# Autodesk Inventor assembly: paddlewheel_assem
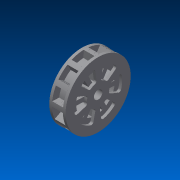
[picture p0: Inventor's stored thumbnail of the model, 180x180]
Saved by Autodesk Inventor 2019 (Build 230136000, 136)
## iProperties
Created: 2018-08-23
Part Number: paddlewheel_assem
Document SubType Name: Assembly
Designer: Kitte_X
Author: Kitte_X
## Documents named in this file (3)
- C:\Users\Kitte_X\Documents\Inventor\paddlewheel_assem.iam
- C:\Users\Kitte_X\Documents\Inventor\paddlewheel_inner.ipt
- C:\Users\Kitte_X\Documents\Inventor\paddlewheel_outer.ipt
## Components (6 placed, 2 different names)
1. paddlewheel_inner:1 — Mate:14, Mate:18, Flush:14, Mate:21, Mate:22
2. paddlewheel_outer:1 — Flush:12, Mate:21, Mate:22, Mate:23, Mate:25, Flush:17
3. paddlewheel_inner:2 — Flush:13, Mate:14, Mate:15, Mate:18, Mate:19, Flush:14, Flush:15
4. paddlewheel_outer:2 — Flush:12, Flush:13, Mate:23, Mate:24
5. paddlewheel_inner:3 — Mate:16, Mate:20, Flush:16, Mate:24
6. paddlewheel_inner:4 — Mate:15, Mate:16, Mate:19, Mate:20, Flush:15, Flush:16
## Relationships (17: Mate 11, Flush 6)
- Flush:12: paddlewheel_outer:1 ↔ paddlewheel_outer:2
- Flush:13: paddlewheel_inner:2 ↔ paddlewheel_outer:2
- Mate:14: paddlewheel_inner:1 ↔ paddlewheel_inner:2
- Mate:15: paddlewheel_inner:2 ↔ paddlewheel_inner:4
- Mate:16: paddlewheel_inner:3 ↔ paddlewheel_inner:4
- Mate:18: paddlewheel_inner:1 ↔ paddlewheel_inner:2
- Mate:19: paddlewheel_inner:2 ↔ paddlewheel_inner:4
- Mate:20: paddlewheel_inner:3 ↔ paddlewheel_inner:4
- Flush:14: paddlewheel_inner:1 ↔ paddlewheel_inner:2
- Flush:15: paddlewheel_inner:2 ↔ paddlewheel_inner:4
- Flush:16: paddlewheel_inner:3 ↔ paddlewheel_inner:4
- Mate:21: paddlewheel_inner:1 ↔ paddlewheel_outer:1
- Mate:22: paddlewheel_inner:1 ↔ paddlewheel_outer:1
- Mate:23: paddlewheel_outer:1 ↔ paddlewheel_outer:2
- Mate:24: paddlewheel_outer:2 ↔ paddlewheel_inner:3
- Mate:25: paddlewheel_outer:1
- Flush:17: paddlewheel_outer:1
